# Autodesk Inventor assembly: main
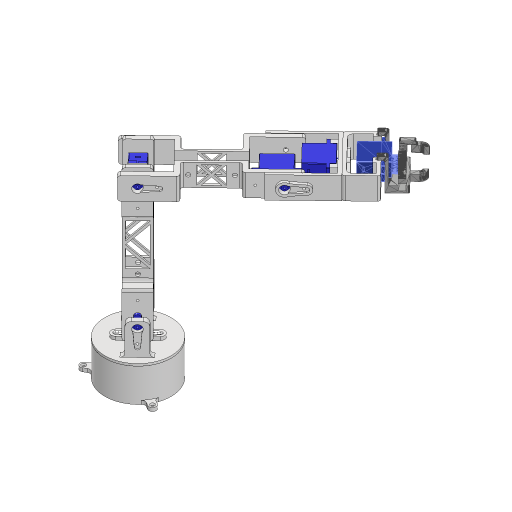
[picture p0: Inventor's stored thumbnail of the model, 512x512]
Saved by Autodesk Inventor 2024.3 (Build 283343000, 343)
## iProperties
Created: 2023-04-29
Part Number: main
Document SubType Name: Assembly
Designer: taka2
Author: taka2
## Documents named in this file (12)
- C:\Users\taka\OneDrive\ドキュメント\04Myproject\Modeling\Inventor\Arm\main.iam
- C:\Users\taka\OneDrive\ドキュメント\04Myproject\Modeling\Inventor\Arm\base.ipt
- C:\Users\taka\OneDrive\ドキュメント\04Myproject\Modeling\Inventor\Arm\base_rot.ipt
- C:\Users\taka\OneDrive\ドキュメント\04Myproject\Modeling\Inventor\template\サーボモータ.ipt
- C:\Users\taka\OneDrive\ドキュメント\04Myproject\Modeling\Inventor\template\サーボホーン.ipt
- C:\Users\taka\OneDrive\ドキュメント\04Myproject\Modeling\Inventor\Arm\joint1_servo.ipt
- C:\Users\taka\OneDrive\ドキュメント\04Myproject\Modeling\Inventor\Arm\joint1_sup.ipt
- C:\Users\taka\OneDrive\ドキュメント\04Myproject\Modeling\Inventor\Arm\joint2_servo.ipt
- C:\Users\taka\OneDrive\ドキュメント\04Myproject\Modeling\Inventor\Arm\joint2_sup.ipt
- C:\Users\taka\OneDrive\ドキュメント\04Myproject\Modeling\Inventor\Arm\joint3.ipt
- C:\Users\taka\OneDrive\ドキュメント\04Myproject\Modeling\Inventor\Arm\joint4.ipt
- C:\Users\taka\OneDrive\ドキュメント\04Myproject\Modeling\Inventor\Arm\Imported Components\endeffector\endeffector.ipt
## Components (15 placed, 11 different names)
1. base:1 — 回転:8, リジッド:1
2. base_rot:1 — 回転:8, リジッド:2, 関節1, 回転:3
3. サーボモータ:1 — リジッド:1
4. サーボホーン:1 — リジッド:2
5. joint1_servo:1 — 関節1, フラッシュ:1, 関節2, リジッド:4, リジッド:5
6. joint1_sup:1 — 回転:3, フラッシュ:1, 回転:5
7. joint2_servo:1 — 関節2, フラッシュ:2, リジッド:6
8. サーボモータ:2 — リジッド:4
9. サーボモータ:3 — リジッド:5
10. joint2_sup:1 — 回転:5, フラッシュ:2
11. joint3:1 — リジッド:11, 関節4, 関節3
12. サーボモータ:4 — リジッド:6, 関節3
13. サーボモータ:5 — リジッド:11
14. joint4:1 — 関節4, リジッド:12
15. endeffector:1 — リジッド:12
## Relationships (16: RevoluteJoint 7, WeldJoint 7, Flush 2)
- 回転:8 [RevoluteJoint]: base:1 ↔ base_rot:1
- リジッド:1 [WeldJoint] (4.5 mm): base:1 ↔ サーボモータ:1
- リジッド:2 [WeldJoint]: base_rot:1 ↔ サーボホーン:1
- 関節1 [RevoluteJoint]: base_rot:1 ↔ joint1_servo:1
- 回転:3 [RevoluteJoint]: base_rot:1 ↔ joint1_sup:1
- フラッシュ:1 [Flush]: joint1_servo:1 ↔ joint1_sup:1
- 関節2 [RevoluteJoint]: joint1_servo:1 ↔ joint2_servo:1
- リジッド:4 [WeldJoint]: joint1_servo:1 ↔ サーボモータ:2
- リジッド:5 [WeldJoint]: joint1_servo:1 ↔ サーボモータ:3
- 回転:5 [RevoluteJoint]: joint1_sup:1 ↔ joint2_sup:1
- フラッシュ:2 [Flush]: joint2_servo:1 ↔ joint2_sup:1
- リジッド:6 [WeldJoint]: joint2_servo:1 ↔ サーボモータ:4
- リジッド:11 [WeldJoint]: joint3:1 ↔ サーボモータ:5
- 関節4 [RevoluteJoint]: joint3:1 ↔ joint4:1
- 関節3 [RevoluteJoint] (-0.5 mm): joint3:1 ↔ サーボモータ:4
- リジッド:12 [WeldJoint]: joint4:1 ↔ endeffector:1
